# Autodesk Inventor assembly: MK3_DriveTrain
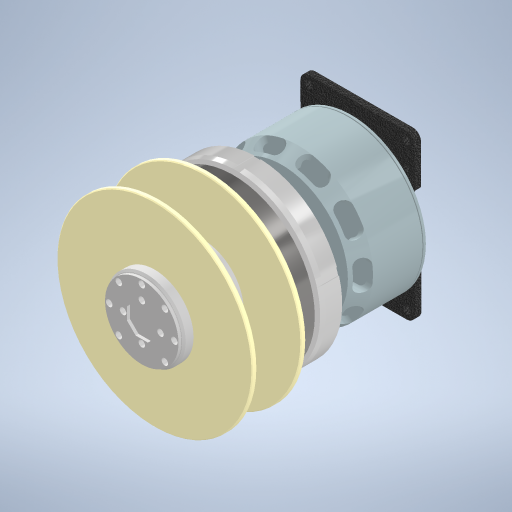
[picture p0: Inventor's stored thumbnail of the model, 512x512]
Saved by Autodesk Inventor 2023.4 (Build 274418000, 418)
## iProperties
Created: 2023-11-23
Part Number: MK3_DriveTrain
Document SubType Name: Assembly
Designer: aaron
Author: aaron
## Documents named in this file (11)
- C:\work\LunarMass\digital_weight_device\cad\v4\drivetrain.iam
- C:\work\LunarMass\digital_weight_device\cad\v4\odrive\100kv_motor.iam
- C:\work\LunarMass\digital_weight_device\cad\v4\motor2_drive_mount.ipt
- C:\work\LunarMass\digital_weight_device\cad\v4\motor2_planetary_gear.ipt
- C:\work\LunarMass\digital_weight_device\cad\v4\motor_mount_plate.ipt
- C:\work\LunarMass\digital_weight_device\cad\v4\planetary_bearing_spacer.ipt
- C:\work\LunarMass\digital_weight_device\cad\bearings\bearing_100x80x10.ipt
- C:\work\LunarMass\digital_weight_device\cad\v4\spool_main_drive.ipt
- C:\work\LunarMass\digital_weight_device\cad\v4\spool_center.ipt
- C:\work\LunarMass\digital_weight_device\cad\v4\spool_side.ipt
- C:\work\LunarMass\digital_weight_device\cad\v4\motor1_drive_mount.ipt
## Components (11 placed, 10 different names)
1. 100kv_motor:1 [sub-assembly] — Insert:1, Insert:3, Insert:4
2. motor2_drive_mount:1 — Insert:1, Insert:2
3. motor2_planetary_gear:1 — Insert:2, Insert:5, Insert:14
4. motor_mount_plate:1 — Insert:3, Insert:4
5. planetary_bearing_spacer:1 — Insert:5, Insert:13
6. bearing_100x80x10:1 — Insert:13, Mate:2
7. spool_main_drive:1 — Insert:14, Mate:1
8. spool_center:1 — Insert:15, Insert:16, Mate:1
9. spool_side:1 — Insert:15, Mate:2
10. spool_side:2 — Insert:16, Insert:17
11. motor1_drive_mount:1 — Insert:17
## Relationships (12: Insert 10, Mate 2)
- Insert:1: 100kv_motor:1 ↔ motor2_drive_mount:1
- Insert:2: motor2_drive_mount:1 ↔ motor2_planetary_gear:1
- Insert:3: 100kv_motor:1 ↔ motor_mount_plate:1
- Insert:4: 100kv_motor:1 ↔ motor_mount_plate:1
- Insert:5: motor2_planetary_gear:1 ↔ planetary_bearing_spacer:1
- Insert:13: planetary_bearing_spacer:1 ↔ bearing_100x80x10:1
- Insert:14: motor2_planetary_gear:1 ↔ spool_main_drive:1
- Insert:15: spool_center:1 ↔ spool_side:1
- Insert:16: spool_center:1 ↔ spool_side:2
- Mate:1: spool_main_drive:1 ↔ spool_center:1
- Mate:2: bearing_100x80x10:1 ↔ spool_side:1
- Insert:17: spool_side:2 ↔ motor1_drive_mount:1
